# Autodesk Inventor assembly: Arm
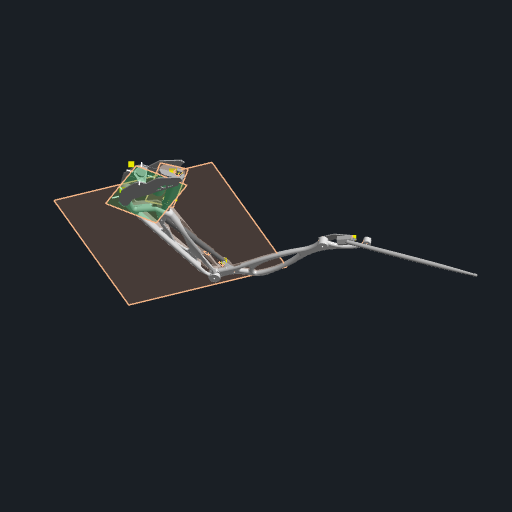
[picture p0: Inventor's stored thumbnail of the model, 512x512]
Saved by Autodesk Inventor 2025.2 (Build 292293000, 293)
## iProperties
Created: 2020-03-24
Part Number: Arm
Document SubType Name: Assembly
Designer: valer
Mass: 4853.13 g
Surface Area: 3141.52 cm^2
Volume: 1403.99 cm^3
Density: 3.45667 g/cm^3
Author: valer
## Documents named in this file (11)
- C:\Users\valer\Desktop\str1ker\cad\Arm.iam
- C:\Users\valer\Desktop\str1ker\cad\UpperArm.iam
- C:\Users\valer\Desktop\str1ker\cad\Forearm.iam
- C:\Users\valer\Desktop\str1ker\cad\ArmSolenoid.iam
- C:\Users\valer\Desktop\str1ker\cad\external\UpperArmActuator\UpperArmActuatorBase.iam
- C:\Users\valer\Desktop\str1ker\cad\external\UpperArmActuator\UpperArmActuatorShaft.iam
- C:\Users\valer\Desktop\str1ker\cad\external\ForearmActuator\ForearmActuatorBody.iam
- C:\Users\valer\Desktop\str1ker\cad\ForearmActuatorConnector.iam
- C:\Users\valer\Desktop\str1ker\cad\external\ForearmActuator\ForearmActuatorShaft.iam
- C:\Users\valer\Desktop\str1ker\cad\Shoulder.iam
- C:\Users\valer\Desktop\str1ker\cad\external\Drumstick\Drumstick.ipt
## Components (10 placed, 10 different names)
1. UpperArm:1 [sub-assembly] — Mate:6, Mate:7, Mate:29, Flush:3, Mate:30, Mate:39, Mate:40
2. Forearm:1 [sub-assembly] — Mate:6, Mate:7, Mate:10, Mate:11, Mate:31
3. ArmSolenoid:1 [sub-assembly] — Mate:10, Mate:11
4. UpperArmActuatorBase:1 [sub-assembly] — Mate:28, Mate:37, Flush:4
5. UpperArmActuatorShaft:1 [sub-assembly] — Mate:28, Mate:29
6. ForearmActuatorBody:1 [sub-assembly] — Flush:3, Mate:30, Mate:32, Mate:33
7. ForearmActuatorConnector:1 [sub-assembly] — Mate:31, Mate:32, Mate:34
8. ForearmActuatorShaft:1 [sub-assembly] — Mate:33, Mate:34
9. Shoulder:1 [sub-assembly] — Mate:37, Mate:39, Mate:40, Flush:4, Mate:41, Angle:1, Angle:2
10. Drumstick:1 — Angle:3
## Relationships (20: Mate 15, Angle 3, Flush 2)
- Mate:6: UpperArm:1 ↔ Forearm:1
- Mate:7: UpperArm:1 ↔ Forearm:1
- Mate:10: Forearm:1 ↔ ArmSolenoid:1
- Mate:11: Forearm:1 ↔ ArmSolenoid:1
- Mate:28: UpperArmActuatorBase:1 ↔ UpperArmActuatorShaft:1
- Mate:29: UpperArm:1 ↔ UpperArmActuatorShaft:1
- Flush:3: UpperArm:1 ↔ ForearmActuatorBody:1
- Mate:30: UpperArm:1 ↔ ForearmActuatorBody:1
- Mate:31: Forearm:1 ↔ ForearmActuatorConnector:1
- Mate:32: ForearmActuatorBody:1 ↔ ForearmActuatorConnector:1
- Mate:33: ForearmActuatorBody:1 ↔ ForearmActuatorShaft:1
- Mate:34: ForearmActuatorConnector:1 ↔ ForearmActuatorShaft:1
- Mate:37: UpperArmActuatorBase:1 ↔ Shoulder:1
- Mate:39: UpperArm:1 ↔ Shoulder:1
- Mate:40: UpperArm:1 ↔ Shoulder:1
- Flush:4 (30.4795 mm): UpperArmActuatorBase:1 ↔ Shoulder:1
- Mate:41: Shoulder:1
- Angle:1 (0 deg): Shoulder:1
- Angle:2 (0 deg): Shoulder:1
- Angle:3 (180 deg): Drumstick:1
